# Autodesk Inventor assembly: HYPNOSIA_6x14
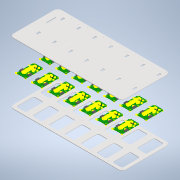
[picture p0: Inventor's stored thumbnail of the model, 180x180]
Saved by Autodesk Inventor 2020 (Build 240168000, 168)
## iProperties
Created: 2020-07-08
Part Number: HYPNOSIA_6x14
Document SubType Name: Assembly
Designer: gerac
Author: gerac
## Documents named in this file (5)
- C:\Users\gerac\Desktop\HES-SO_3\BACHELOR_THESIS\HypnosiaControllerGIT\HYPNOSIA_Inventor\HYPNOSIA_6x14.iam
- HYPNOSIA_6x14.iam
- C:\Users\gerac\Desktop\HES-SO_3\BACHELOR_THESIS\HypnosiaControllerGIT\HYPNOSIA_Inventor\HYPNOSIA_V2.iam
- C:\Users\gerac\Desktop\HES-SO_3\BACHELOR_THESIS\HypnosiaControllerGIT\HYPNOSIA_Inventor\back_Box.ipt
- C:\Users\gerac\Desktop\HES-SO_3\BACHELOR_THESIS\HypnosiaControllerGIT\HYPNOSIA_Inventor\front_Box.ipt
## Components (16 placed, 3 different names)
1. back_Box:1 — Flush:1, Flush:2, Flush:3, Mate:2, Mate:3
2. front_Box:1 — Flush:2, Flush:3
3. HYPNOSIA_V2:1 [sub-assembly]
4. HYPNOSIA_V2:2 [sub-assembly] — Mate:1
5. HYPNOSIA_V2:3 [sub-assembly]
6. HYPNOSIA_V2:4 [sub-assembly]
7. HYPNOSIA_V2:5 [sub-assembly]
8. HYPNOSIA_V2:6 [sub-assembly]
9. HYPNOSIA_V2:7 [sub-assembly]
10. HYPNOSIA_V2:8 [sub-assembly]
11. HYPNOSIA_V2:9 [sub-assembly]
12. HYPNOSIA_V2:10 [sub-assembly]
13. HYPNOSIA_V2:11 [sub-assembly]
14. HYPNOSIA_V2:12 [sub-assembly]
15. HYPNOSIA_V2:13 [sub-assembly]
16. HYPNOSIA_V2:14 [sub-assembly] — Mate:2, Mate:3
## Component patterns: (14 elements, first: HYPNOSIA_V2:1)
## Relationships (6: Mate 3, Flush 3)
- Mate:1: HYPNOSIA_V2:2
- Flush:1: back_Box:1
- Flush:2: back_Box:1 ↔ front_Box:1
- Flush:3: back_Box:1 ↔ front_Box:1
- Mate:2: back_Box:1 ↔ HYPNOSIA_V2:14
- Mate:3: back_Box:1 ↔ HYPNOSIA_V2:14
